# Autodesk Inventor assembly: airhockeybot_y_simulation
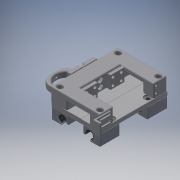
[picture p0: Inventor's stored thumbnail of the model, 180x180]
Saved by Autodesk Inventor 2019.3 (Build 233278000, 278)
## iProperties
Created: 2020-08-23
Part Number: airhockeybot_y_simulation
Material: Generisch
Document SubType Name: Assembly
Designer: Nicolas Frick
Author: Nicolas Frick
## Documents named in this file (6)
- C:\Users\Nicolas Frick\Sync\OneDrive\airhockeybot\mechanical_design\common_cad_parts\sim_models\airhockeybot_y_simulation.iam
- C:\Users\Nicolas Frick\Sync\OneDrive\airhockeybot\mechanical_design\inventor\igus\Schlitten_WW_10_40_10_1.ipt
- C:\Users\Nicolas Frick\Sync\OneDrive\airhockeybot\mechanical_design\inventor\Bat_fixture.ipt
- C:\Users\Nicolas Frick\Sync\OneDrive\airhockeybot\mechanical_design\inventor\MaedlerKlemmplatte_T2_5_6mm\16069900.ipt
- C:\Users\Nicolas Frick\Sync\OneDrive\airhockeybot\mechanical_design\inventor\Bat_claw.ipt
- C:\Users\Nicolas Frick\Sync\OneDrive\airhockeybot\mechanical_design\inventor\Pusher.ipt
## Components (6 placed, 5 different names)
1. Schlitten_WW_10_40_10_1:1 — Fluchtend:64, Passend:179, Passend:180, Passend:181, Passend:182
2. Bat_fixture:1 — Fluchtend:64, Fluchtend:65, Fluchtend:67, Fluchtend:68, Passend:178, Passend:181, Passend:182, Fluchtend:69, Fluchtend:70, Passend:185, Fluchtend:77, Fluchtend:85, Fluchtend:86
3. 16069900:1 — Fluchtend:65, Fluchtend:67, Passend:180
4. 16069900:2 — Fluchtend:68, Passend:178, Passend:179
5. Bat_claw:1 — Fluchtend:69, Fluchtend:70, Passend:185
6. Pusher:1 — Fluchtend:77, Fluchtend:85, Fluchtend:86
## Relationships (15: Flush 9, Mate 6)
- Fluchtend:64 [Flush]: Schlitten_WW_10_40_10_1:1 ↔ Bat_fixture:1
- Fluchtend:65 [Flush] (-5.5 mm): Bat_fixture:1 ↔ 16069900:1
- Fluchtend:67 [Flush] (20 mm): Bat_fixture:1 ↔ 16069900:1
- Fluchtend:68 [Flush] (-5.5 mm): Bat_fixture:1 ↔ 16069900:2
- Passend:178 [Mate]: Bat_fixture:1 ↔ 16069900:2
- Passend:179 [Mate]: Schlitten_WW_10_40_10_1:1 ↔ 16069900:2
- Passend:180 [Mate]: Schlitten_WW_10_40_10_1:1 ↔ 16069900:1
- Passend:181 [Mate]: Schlitten_WW_10_40_10_1:1 ↔ Bat_fixture:1
- Passend:182 [Mate]: Schlitten_WW_10_40_10_1:1 ↔ Bat_fixture:1
- Fluchtend:69 [Flush] (30 mm): Bat_fixture:1 ↔ Bat_claw:1
- Fluchtend:70 [Flush]: Bat_fixture:1 ↔ Bat_claw:1
- Passend:185 [Mate]: Bat_fixture:1 ↔ Bat_claw:1
- Fluchtend:77 [Flush]: Bat_fixture:1 ↔ Pusher:1
- Fluchtend:85 [Flush] (-10 mm): Bat_fixture:1 ↔ Pusher:1
- Fluchtend:86 [Flush] (2 mm): Bat_fixture:1 ↔ Pusher:1
